# Autodesk Inventor assembly: omni
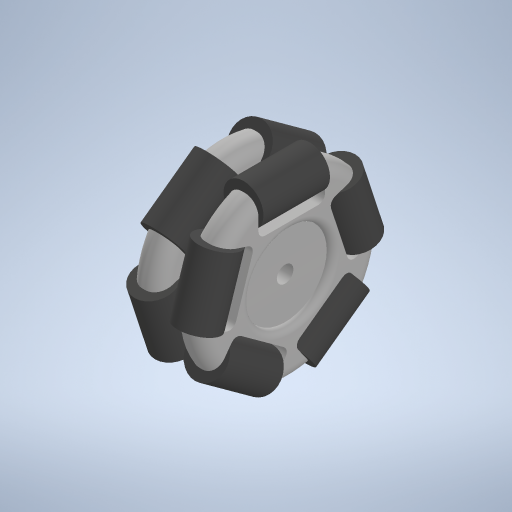
[picture p0: Inventor's stored thumbnail of the model, 512x512]
Saved by Autodesk Inventor 2024.1 (Build 281209000, 209)
## iProperties
Created: 2024-08-02
Part Number: omni
Document SubType Name: Assembly
Designer: hibik
Author: hibik
## Documents named in this file (2)
- C:\Users\hibik\Desktop\ロボメカ\Rescue\2年\子機_本選\omni.iam
- C:\Users\hibik\Desktop\ロボメカ\Rescue\2年\子機_本選\omni_half.ipt
## Components (2 placed, 1 different names)
1. omni_half:1 — 挿入:1, 角度:1
2. omni_half:2 — 挿入:1, 角度:1
## Relationships (2: Insert 1, Angle 1)
- 挿入:1 [Insert]: omni_half:1 ↔ omni_half:2
- 角度:1 [Angle] (36 deg): omni_half:1 ↔ omni_half:2
